# Autodesk Inventor assembly: Motor_64
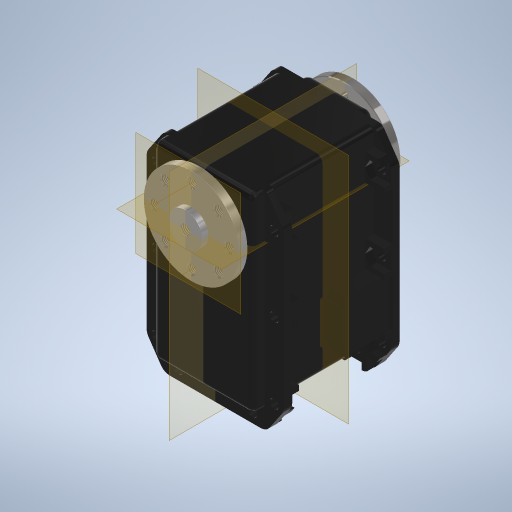
[picture p0: Inventor's stored thumbnail of the model, 512x512]
Saved by Autodesk Inventor 2024.3 (Build 283343000, 343)
## iProperties
Created: 2024-09-05
Part Number: Motor_64
Document SubType Name: Assembly
Designer: gretc
Author: gretc
## Documents named in this file (4)
- C:\Users\gretc\Desktop\inventor_part\Motor_64.iam
- C:\Users\gretc\Desktop\inventor_part\혼\64-106Horn.ipt
- C:\Users\gretc\Desktop\inventor_part\다이나믹셀\MX-64T+idle.ipt.iam
- MX-64T+idle.ipt
## Components (2 placed, 2 different names)
1. 64-106Horn:1 — 삽입:1
2. MX-64T+idle.ipt:1 [sub-assembly] — 삽입:1
## Relationships (1: Insert 1)
- 삽입:1 [Insert] (0.5 mm): 64-106Horn:1 ↔ MX-64T+idle.ipt:1
